# Autodesk Inventor assembly: A2017_T4_01
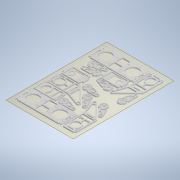
[picture p0: Inventor's stored thumbnail of the model, 180x180]
Saved by Autodesk Inventor 2020 (Build 240168000, 168)
## iProperties
Created: 2021-08-27
Part Number: A2017_T4_01
Document SubType Name: Assembly
Designer: Masato
Author: Masato
## Documents named in this file (9)
- C:\Users\naoki\Documents\Inventor\CitBrains\git_clone\SUSTAINA_ver1_0\AT4_02\SUSTAINA-OP\Cam\A2017_T4_01.iam
- C:\Users\naoki\Documents\Inventor\CitBrains\git_clone\SUSTAINA_ver1_0\AT4_172\SUSTAINA-OP\Cam\DisposableBoard.ipt
- C:\Users\naoki\Documents\Inventor\CitBrains\git_clone\SUSTAINA_ver1_0\AT4_172\SUSTAINA-OP\LowerBody\Ankle\Ankle_side_pitch_frame.ipt
- C:\Users\naoki\Documents\Inventor\CitBrains\git_clone\SUSTAINA_ver1_0\AT4_172\SUSTAINA-OP\UpperBody\Trunk\Trunk_neck_frame.ipt
- C:\Users\naoki\Documents\Inventor\CitBrains\git_clone\SUSTAINA_ver1_0\AT4_172\SUSTAINA-OP\UpperBody\Trunk\Trunk_shoulder_frame.ipt
- C:\Users\naoki\Documents\Inventor\CitBrains\git_clone\SUSTAINA_ver1_0\AT4_172\SUSTAINA-OP\UpperBody\Trunk\Trunk_shoulder_frame_MIR.ipt
- C:\Users\naoki\Documents\Inventor\CitBrains\git_clone\SUSTAINA_ver1_0\AT4_172\SUSTAINA-OP\UpperBody\Trunk\Trunk_waisit_frame.ipt
- C:\Users\naoki\Documents\Inventor\CitBrains\git_clone\SUSTAINA_ver1_0\AT4_172\SUSTAINA-OP\UpperBody\Trunk\Trunk_servo_bottom_frame.ipt
- C:\Users\naoki\Documents\Inventor\CitBrains\git_clone\SUSTAINA_ver1_0\AT4_02\SUSTAINA-OP\UpperBody\Trunk\Trunk_servo_bottom_frame.ipt
## Components (17 placed, 7 different names)
1. DisposableBoard:1 — メイト:2, メイト:1, フラッシュ:1, フラッシュ:2, フラッシュ:3, フラッシュ:5, メイト:22, メイト:24, フラッシュ:8, フラッシュ:9, フラッシュ:10, フラッシュ:11, メイト:27, メイト:28, メイト:29, 角度:1, メイト:32, 角度:2, メイト:37, メイト:38, メイト:41
2. Trunk_neck_frame:1 — メイト:6, フラッシュ:6, フラッシュ:7, メイト:16, メイト:17, 正接:2
3. Trunk_shoulder_frame:1 — メイト:9, フラッシュ:4, メイト:15, メイト:21, 正接:3, 正接:4
4. Trunk_shoulder_frame_MIR:1 — メイト:10, フラッシュ:7, メイト:17, メイト:20, 正接:10
5. Trunk_waisit_frame:1 — フラッシュ:3, フラッシュ:4, フラッシュ:5, フラッシュ:6, メイト:15, メイト:16, メイト:19
6. Ankle_side_pitch_frame:2 — メイト:5, メイト:19, 正接:2
7. Ankle_side_pitch_frame:1 — メイト:4, メイト:20, 正接:3, 正接:9
8. Trunk_servo_bottom_frame:2 — メイト:14
9. Ankle_side_pitch_frame:3 — メイト:21, メイト:22, 正接:4
10. Trunk_waisit_frame:2 — フラッシュ:10, メイト:27, メイト:30, メイト:39, メイト:42
11. Trunk_shoulder_frame_MIR:2 — メイト:24, 正接:5, フラッシュ:9, フラッシュ:11, メイト:30, 正接:7, メイト:43
12. Ankle_side_pitch_frame:4 — フラッシュ:8, 正接:5, メイト:32
13. Ankle_side_pitch_frame:6 — メイト:29, 正接:7, 角度:1
14. Ankle_side_pitch_frame:7 — メイト:28, 正接:9, 正接:10, 角度:2
15. Ankle_side_pitch_frame:8 — メイト:37, メイト:39, メイト:40, 正接:11
16. Ankle_side_pitch_frame:9 — メイト:38, メイト:40
17. Trunk_servo_bottom_frame:3 — メイト:41, メイト:42, 正接:11, メイト:43
## Relationships (49: Mate 28, Flush 11, Tangent 8, Angle 2)
- メイト:2 [Mate]: DisposableBoard:1
- メイト:1 [Mate]: DisposableBoard:1
- フラッシュ:1 [Flush]: DisposableBoard:1
- フラッシュ:2 [Flush]: DisposableBoard:1
- メイト:4 [Mate]: Ankle_side_pitch_frame:1
- メイト:5 [Mate]: Ankle_side_pitch_frame:2
- メイト:6 [Mate]: Trunk_neck_frame:1
- メイト:9 [Mate]: Trunk_shoulder_frame:1
- メイト:10 [Mate]: Trunk_shoulder_frame_MIR:1
- メイト:14 [Mate]: Trunk_servo_bottom_frame:2
- フラッシュ:3 [Flush] (2 mm): DisposableBoard:1 ↔ Trunk_waisit_frame:1
- フラッシュ:4 [Flush]: Trunk_shoulder_frame:1 ↔ Trunk_waisit_frame:1
- フラッシュ:5 [Flush] (2 mm): DisposableBoard:1 ↔ Trunk_waisit_frame:1
- フラッシュ:6 [Flush]: Trunk_neck_frame:1 ↔ Trunk_waisit_frame:1
- フラッシュ:7 [Flush]: Trunk_neck_frame:1 ↔ Trunk_shoulder_frame_MIR:1
- メイト:15 [Mate] (2.5 mm): Trunk_shoulder_frame:1 ↔ Trunk_waisit_frame:1
- メイト:16 [Mate] (2.5 mm): Trunk_neck_frame:1 ↔ Trunk_waisit_frame:1
- メイト:17 [Mate] (2.5 mm): Trunk_neck_frame:1 ↔ Trunk_shoulder_frame_MIR:1
- メイト:19 [Mate] (2.5 mm): Trunk_waisit_frame:1 ↔ Ankle_side_pitch_frame:2
- メイト:20 [Mate] (2.5 mm): Trunk_shoulder_frame_MIR:1 ↔ Ankle_side_pitch_frame:1
- メイト:21 [Mate] (2.5 mm): Trunk_shoulder_frame:1 ↔ Ankle_side_pitch_frame:3
- メイト:22 [Mate]: DisposableBoard:1 ↔ Ankle_side_pitch_frame:3
- 正接:2 [Tangent] (2.5 mm): Trunk_neck_frame:1 ↔ Ankle_side_pitch_frame:2
- 正接:3 [Tangent] (2.5 mm): Trunk_shoulder_frame:1 ↔ Ankle_side_pitch_frame:1
- 正接:4 [Tangent] (1 mm): Trunk_shoulder_frame:1 ↔ Ankle_side_pitch_frame:3
- メイト:24 [Mate]: DisposableBoard:1 ↔ Trunk_shoulder_frame_MIR:2
- フラッシュ:8 [Flush] (2.5 mm): DisposableBoard:1 ↔ Ankle_side_pitch_frame:4
- 正接:5 [Tangent] (2.5 mm): Trunk_shoulder_frame_MIR:2 ↔ Ankle_side_pitch_frame:4
- フラッシュ:9 [Flush] (2 mm): DisposableBoard:1 ↔ Trunk_shoulder_frame_MIR:2
- フラッシュ:10 [Flush] (2 mm): DisposableBoard:1 ↔ Trunk_waisit_frame:2
- フラッシュ:11 [Flush] (2 mm): DisposableBoard:1 ↔ Trunk_shoulder_frame_MIR:2
- メイト:27 [Mate]: DisposableBoard:1 ↔ Trunk_waisit_frame:2
- メイト:28 [Mate]: DisposableBoard:1 ↔ Ankle_side_pitch_frame:7
- メイト:29 [Mate]: DisposableBoard:1 ↔ Ankle_side_pitch_frame:6
- メイト:30 [Mate] (2.5 mm): Trunk_waisit_frame:2 ↔ Trunk_shoulder_frame_MIR:2
- 正接:7 [Tangent] (2.5 mm): Trunk_shoulder_frame_MIR:2 ↔ Ankle_side_pitch_frame:6
- 角度:1 [Angle] (0 deg): DisposableBoard:1 ↔ Ankle_side_pitch_frame:6
- メイト:32 [Mate]: DisposableBoard:1 ↔ Ankle_side_pitch_frame:4
- 正接:9 [Tangent] (2.5 mm): Ankle_side_pitch_frame:1 ↔ Ankle_side_pitch_frame:7
- 正接:10 [Tangent] (2.5 mm): Trunk_shoulder_frame_MIR:1 ↔ Ankle_side_pitch_frame:7
- 角度:2 [Angle] (0 deg): DisposableBoard:1 ↔ Ankle_side_pitch_frame:7
- メイト:37 [Mate]: DisposableBoard:1 ↔ Ankle_side_pitch_frame:8
- メイト:38 [Mate]: DisposableBoard:1 ↔ Ankle_side_pitch_frame:9
- メイト:39 [Mate] (2.5 mm): Trunk_waisit_frame:2 ↔ Ankle_side_pitch_frame:8
- メイト:40 [Mate] (2.5 mm): Ankle_side_pitch_frame:8 ↔ Ankle_side_pitch_frame:9
- メイト:41 [Mate]: DisposableBoard:1 ↔ Trunk_servo_bottom_frame:3
- メイト:42 [Mate] (2.5 mm): Trunk_waisit_frame:2 ↔ Trunk_servo_bottom_frame:3
- 正接:11 [Tangent] (2.5 mm): Ankle_side_pitch_frame:8 ↔ Trunk_servo_bottom_frame:3
- メイト:43 [Mate] (2.5 mm): Trunk_shoulder_frame_MIR:2 ↔ Trunk_servo_bottom_frame:3
